# Autodesk Inventor assembly: Module without cover
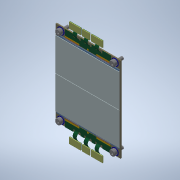
[picture p0: Inventor's stored thumbnail of the model, 180x180]
Saved by Autodesk Inventor 2022 (Build 260153000, 153)
## iProperties
Created: 2021-01-15
Part Number: Module without cover
Document SubType Name: Assembly
Designer: caleb
Author: caleb
## Documents named in this file (10)
- C:\Users\Caleb\Desktop\nebraska-silicon-lab\Hardware\ETL\modules\tdr\Module without cover.iam
- C:\Users\Caleb\Desktop\nebraska-silicon-lab\Hardware\ETL\modules\tdr\F10109317--_1-MODULE_ CMS2 ETL_ FLEX CIRCUIT.ipt
- C:\Users\Caleb\Desktop\nebraska-silicon-lab\Hardware\ETL\modules\tdr\F10109316--_1-MODULE_ CMS2 ETL_ ALN SUBSTRATE.ipt
- C:\Users\Caleb\Desktop\nebraska-silicon-lab\Hardware\ETL\modules\tdr\F10109315--_1-LAYOUT_ CMS2 ETL MODULE CONCEPT_ SEP-2018 SENSOR SUBASSY_MODEL.iam
- C:\Users\Caleb\Desktop\nebraska-silicon-lab\Hardware\ETL\modules\tdr\F10110221--_1-MODULE_ CMS2 ETL_ FLEX CIRCUIT WIREBONDS.ipt
- C:\Users\Caleb\Desktop\nebraska-silicon-lab\Hardware\ETL\modules\tdr\F10112322--_1-MODULE_ CMS2 ETL_ READOUT CHIP MOUNTING FILM.ipt
- C:\Users\Caleb\Desktop\nebraska-silicon-lab\Hardware\ETL\modules\tdr\F10112323--_1-MODULE_ CMS2 ETL_ FLEX CIRCUIT MOUNTING FILM.ipt
- C:\Users\Caleb\Desktop\nebraska-silicon-lab\Hardware\ETL\modules\tdr\F10110888--_1-MODULE_ CMS2 ETL_ SUBSTRATE MOUNTING THERMAL PAD.ipt
- C:\Users\Caleb\Desktop\nebraska-silicon-lab\Hardware\ETL\modules\tdr\FC0041908--_1-SHCS_M2x.4x5LGxFT_SS316L_ROLLED_EP.ipt
- C:\Users\Caleb\Desktop\nebraska-silicon-lab\Hardware\ETL\modules\tdr\F10109326--_1-WASHER_ BELLEVILLE_ .093IDx.187ODx.01THK_ 17-7 PH STAINLESS STEEL.ipt
## Components (19 placed, 13 different names)
1. F10109317--_1-MODULE_ CMS2 ETL_ FLEX CIRCUIT_1005
2. F10109316--_1-MODULE_ CMS2 ETL_ ALN SUBSTRATE_1006 — Insert:1, Insert:2, Insert:3, Insert:4
3. F10109315--_1-LAYOUT_ CMS2 ETL MODULE CONCEPT_ SEP-2018 SENSOR SUBASSY_MODEL_1007 [sub-assembly]
4. F10110221--_1-MODULE_ CMS2 ETL_ FLEX CIRCUIT WIREBONDS_1008
5. F10109315--_1-LAYOUT_ CMS2 ETL MODULE CONCEPT_ SEP-2018 SENSOR SUBASSY_MODEL_1009 [sub-assembly]
6. F10112322--_1-MODULE_ CMS2 ETL_ READOUT CHIP MOUNTING FILM_1010
7. F10112323--_1-MODULE_ CMS2 ETL_ FLEX CIRCUIT MOUNTING FILM_1011
8. F10110888--_1-MODULE_ CMS2 ETL_ SUBSTRATE MOUNTING THERMAL PAD_1012
9. F10109317--_1-MODULE_ CMS2 ETL_ FLEX CIRCUIT_1013
10. F10112323--_1-MODULE_ CMS2 ETL_ FLEX CIRCUIT MOUNTING FILM_1014
11. F10110221--_1-MODULE_ CMS2 ETL_ FLEX CIRCUIT WIREBONDS_1017
12. FC0041908--_1-SHCS_M2x.4x5LGxFT_SS316L_ROLLED_EP:1 — Insert:5
13. FC0041908--_1-SHCS_M2x.4x5LGxFT_SS316L_ROLLED_EP:2 — Insert:6
14. FC0041908--_1-SHCS_M2x.4x5LGxFT_SS316L_ROLLED_EP:3 — Insert:7
15. FC0041908--_1-SHCS_M2x.4x5LGxFT_SS316L_ROLLED_EP:4 — Insert:8
16. F10109326--_1-WASHER_ BELLEVILLE_ .093IDx.187ODx.01THK_ 17-7 PH STAINLESS STEEL:1 — Insert:1, Insert:5
17. F10109326--_1-WASHER_ BELLEVILLE_ .093IDx.187ODx.01THK_ 17-7 PH STAINLESS STEEL:2 — Insert:2, Insert:6
18. F10109326--_1-WASHER_ BELLEVILLE_ .093IDx.187ODx.01THK_ 17-7 PH STAINLESS STEEL:3 — Insert:3, Insert:7
19. F10109326--_1-WASHER_ BELLEVILLE_ .093IDx.187ODx.01THK_ 17-7 PH STAINLESS STEEL:4 — Insert:4, Insert:8
## Relationships (8: Insert 8)
- Insert:1: F10109316--_1-MODULE_ CMS2 ETL_ ALN SUBSTRATE_1006 ↔ F10109326--_1-WASHER_ BELLEVILLE_ .093IDx.187ODx.01THK_ 17-7 PH STAINLESS STEEL:1
- Insert:2: F10109316--_1-MODULE_ CMS2 ETL_ ALN SUBSTRATE_1006 ↔ F10109326--_1-WASHER_ BELLEVILLE_ .093IDx.187ODx.01THK_ 17-7 PH STAINLESS STEEL:2
- Insert:3: F10109316--_1-MODULE_ CMS2 ETL_ ALN SUBSTRATE_1006 ↔ F10109326--_1-WASHER_ BELLEVILLE_ .093IDx.187ODx.01THK_ 17-7 PH STAINLESS STEEL:3
- Insert:4: F10109316--_1-MODULE_ CMS2 ETL_ ALN SUBSTRATE_1006 ↔ F10109326--_1-WASHER_ BELLEVILLE_ .093IDx.187ODx.01THK_ 17-7 PH STAINLESS STEEL:4
- Insert:5: FC0041908--_1-SHCS_M2x.4x5LGxFT_SS316L_ROLLED_EP:1 ↔ F10109326--_1-WASHER_ BELLEVILLE_ .093IDx.187ODx.01THK_ 17-7 PH STAINLESS STEEL:1
- Insert:6: FC0041908--_1-SHCS_M2x.4x5LGxFT_SS316L_ROLLED_EP:2 ↔ F10109326--_1-WASHER_ BELLEVILLE_ .093IDx.187ODx.01THK_ 17-7 PH STAINLESS STEEL:2
- Insert:7: FC0041908--_1-SHCS_M2x.4x5LGxFT_SS316L_ROLLED_EP:3 ↔ F10109326--_1-WASHER_ BELLEVILLE_ .093IDx.187ODx.01THK_ 17-7 PH STAINLESS STEEL:3
- Insert:8: FC0041908--_1-SHCS_M2x.4x5LGxFT_SS316L_ROLLED_EP:4 ↔ F10109326--_1-WASHER_ BELLEVILLE_ .093IDx.187ODx.01THK_ 17-7 PH STAINLESS STEEL:4
